# Autodesk Inventor assembly: cpu
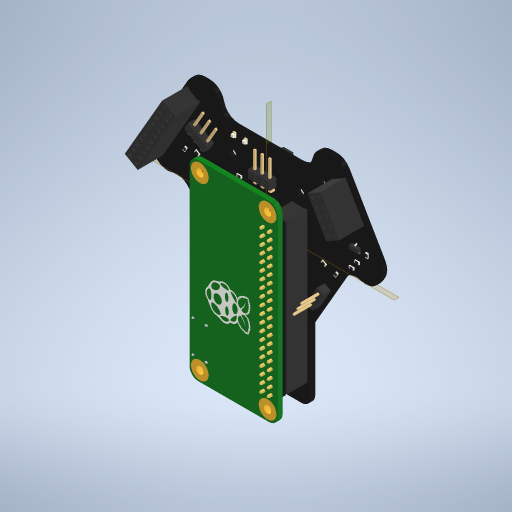
[picture p0: Inventor's stored thumbnail of the model, 512x512]
Saved by Autodesk Inventor 2024.1 (Build 281209000, 209)
## iProperties
Company: Kicad
Created: 2025-04-21
Part Number: cpu
Description: KiCad electronic assembly
Document SubType Name: Assembly
Designer: hibik
Authority: Unknown
Sending System: KiCad to STEP converter
Preprocessor: Open CASCADE STEP processor 7.8
Title: core_assy.step
Author: Pcbnew
## Documents named in this file (16)
- C:\Users\hibik\Documents\Robomech\RESCUE\ORCA\hard\board\CORE_model\cpu.iam
- C:\Users\hibik\Documents\Robomech\RESCUE\ORCA\hard\board\core_assy\R_0603_1608Metric.ipt
- C:\Users\hibik\Documents\Robomech\RESCUE\ORCA\hard\board\core_assy\LED_0603_1608Metric.ipt
- C:\Users\hibik\Documents\Robomech\RESCUE\ORCA\hard\board\core_assy\PinHeader_1x03_P2.54mm_Horizontal.ipt
- C:\Users\hibik\Documents\Robomech\RESCUE\ORCA\hard\board\core_assy\Raspberry_PI_Zero_W.iam
- C:\Users\hibik\Documents\Robomech\RESCUE\ORCA\hard\board\core_assy\PinSocket_2x20_P2.54mm_Vertical.ipt
- C:\Users\hibik\Documents\Robomech\RESCUE\ORCA\hard\board\core_assy\C_1206_3216Metric.ipt
- C:\Users\hibik\Documents\Robomech\RESCUE\ORCA\hard\board\core_assy\SOT-23.ipt
- C:\Users\hibik\Documents\Robomech\RESCUE\ORCA\hard\board\core_assy\C_0603_1608Metric.ipt
- C:\Users\hibik\Documents\Robomech\RESCUE\ORCA\hard\board\core_assy\PMW3360.iam
- C:\Users\hibik\Documents\Robomech\RESCUE\ORCA\hard\board\core_assy\PinHeader_1x03_P2.54mm_Vertical.ipt
- C:\Users\hibik\Documents\Robomech\RESCUE\ORCA\hard\board\core_assy\PinSocket_2x10_P2.54mm_Vertical.ipt
- C:\Users\hibik\Documents\Robomech\RESCUE\ORCA\hard\board\core_assy\PinSocket_2x05_P2.54mm_Vertical.ipt
- C:\Users\hibik\Documents\Robomech\RESCUE\ORCA\hard\board\core_assy\C_0805_2012Metric.ipt
- C:\Users\hibik\Documents\Robomech\RESCUE\ORCA\hard\board\core_assy\SOT-223.ipt
- C:\Users\hibik\Documents\Robomech\RESCUE\ORCA\hard\board\core_assy\ORCA_CORE_PCB_1.ipt
## Components (55 placed, 55 different names)
1. 2
2. 6
3. 8
4. 12
5. 13
6. 14
7. 136 [sub-assembly]
8. 137
9. 152
10. 157
11. 160
12. 164
13. 165
14. 166
15. 167
16. 169
17. 174
18. 175
19. 195 [sub-assembly]
20. 196
21. 198
22. 202
23. 207
24. 209
25. 211
26. 212
27. 214
28. 215
29. 222
30. 227
31. 228
32. 230
33. 232
34. 236
35. 239
36. 241
37. 244
38. 245
39. 246
40. 247
41. 250
42. 253
43. 255
44. 257
45. 259
46. 270
47. 275
48. 278
49. 290
50. 295
51. 299
52. 300
53. 301
54. 304
55. 306 — フラッシュ:1, フラッシュ:2
## Relationships (2: Flush 2)
- フラッシュ:1 [Flush] (4.27 mm): 306
- フラッシュ:2 [Flush] (-24.01 mm): 306
